# Autodesk Inventor assembly: AssembledParts
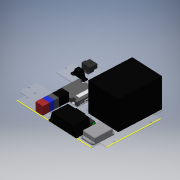
[picture p0: Inventor's stored thumbnail of the model, 180x180]
Saved by Autodesk Inventor 2017 (Build 210142000, 142)
## iProperties
Created: 2017-02-10
Part Number: AssembledParts
Document SubType Name: Assembly
Designer: michael
Author: michael
## Documents named in this file (12)
- C:\Users\michael\Documents\Jinx\AssembledParts.iam
- C:\Users\michael\Documents\Jinx\Parts\Base.ipt
- C:\Users\michael\Documents\Jinx\Parts\Computer.ipt
- C:\Users\michael\Documents\Jinx\Parts\RoboteQ MDC2460.ipt
- C:\Users\michael\Documents\Jinx\Parts\1047_1.ipt
- C:\Users\michael\Documents\Jinx\Parts\24v Converter.ipt
- C:\Users\michael\Documents\Jinx\Parts\12v_dc_to_dc.ipt
- C:\Users\michael\Documents\Jinx\Parts\TerminalBlock.iam
- C:\Users\michael\Documents\Jinx\Parts\relays.ipt
- C:\Users\michael\Documents\Jinx\Parts\Fuse Block.ipt
- C:\Users\michael\Documents\Jinx\Parts\BatteryVoltage.ipt
- C:\Users\michael\Documents\Jinx\Parts\5v dc to dc\pyb15-q24-s5-t.iam
## Components (11 placed, 11 different names)
1. Base:1 — Mate:1, Mate:2, Mate:3, Mate:4, Mate:5, Mate:20, Mate:21, Mate:22, Mate:29, Mate:30, Mate:31, Mate:32, Mate:33, Mate:34, Mate:35, Mate:36, Mate:37, Mate:38, Mate:39, Mate:40, Mate:41, Mate:42, Mate:43, Mate:50, Mate:51, Mate:52, Mate:53, Mate:54, Mate:55
2. Computer:1 — Mate:1, Mate:2
3. RoboteQ MDC2460:1 — Mate:3, Mate:4, Mate:5
4. relays:1 — Mate:20, Mate:21, Mate:22
5. Fuse Block:1 — Mate:29, Mate:30, Mate:31
6. BatteryVoltage:1 — Mate:32, Mate:33, Mate:34
7. 12v_dc_to_dc:1 — Mate:38, Mate:39, Mate:40
8. 24v Converter:1 — Mate:41, Mate:42, Mate:43
9. TerminalBlock:1 [sub-assembly] — Mate:35, Mate:36, Mate:37
10. pyb15-q24-s5-t:1 [sub-assembly] — Mate:50, Mate:51, Mate:52
11. 1047_1:1 — Mate:53, Mate:54, Mate:55
## Relationships (29: Mate 29)
- Mate:1 (50.8 mm): Base:1 ↔ Computer:1
- Mate:2: Base:1 ↔ Computer:1
- Mate:3: Base:1 ↔ RoboteQ MDC2460:1
- Mate:4: Base:1 ↔ RoboteQ MDC2460:1
- Mate:5: Base:1 ↔ RoboteQ MDC2460:1
- Mate:20: Base:1 ↔ relays:1
- Mate:21: Base:1 ↔ relays:1
- Mate:22: Base:1 ↔ relays:1
- Mate:29: Base:1 ↔ Fuse Block:1
- Mate:30: Base:1 ↔ Fuse Block:1
- Mate:31: Base:1 ↔ Fuse Block:1
- Mate:32: Base:1 ↔ BatteryVoltage:1
- Mate:33: Base:1 ↔ BatteryVoltage:1
- Mate:34: Base:1 ↔ BatteryVoltage:1
- Mate:35: Base:1 ↔ TerminalBlock:1
- Mate:36: Base:1 ↔ TerminalBlock:1
- Mate:37: Base:1 ↔ TerminalBlock:1
- Mate:38: Base:1 ↔ 12v_dc_to_dc:1
- Mate:39: Base:1 ↔ 12v_dc_to_dc:1
- Mate:40: Base:1 ↔ 12v_dc_to_dc:1
- Mate:41: Base:1 ↔ 24v Converter:1
- Mate:42: Base:1 ↔ 24v Converter:1
- Mate:43: Base:1 ↔ 24v Converter:1
- Mate:50: Base:1 ↔ pyb15-q24-s5-t:1
- Mate:51: Base:1 ↔ pyb15-q24-s5-t:1
- Mate:52: Base:1 ↔ pyb15-q24-s5-t:1
- Mate:53: Base:1 ↔ 1047_1:1
- Mate:54: Base:1 ↔ 1047_1:1
- Mate:55: Base:1 ↔ 1047_1:1
